# Autodesk Inventor assembly: LEFT RAIL ASSY
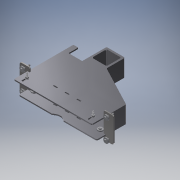
[picture p0: Inventor's stored thumbnail of the model, 180x180]
Saved by Autodesk Inventor 2018 (Build 220112000, 112)
## iProperties
Created: 2018-10-15
Part Number: LEFT RAIL ASSY
Material: Genérico
Document SubType Name: Assembly
Designer: Toshiba
Author: Toshiba
## Documents named in this file (7)
- C:\U\Semestre Primavera 2018\Diseño de sistemas mecánicos\CNC\DiseñoCNC\Gantry\LEFT RAIL ASSY.iam
- C:\U\Semestre Primavera 2018\Diseño de sistemas mecánicos\CNC\DiseñoCNC\Gantry\INTERNAL SIDE PLATE.ipt
- C:\U\Semestre Primavera 2018\Diseño de sistemas mecánicos\CNC\DiseñoCNC\Gantry\INTERNAL FRAME.ipt
- C:\U\Semestre Primavera 2018\Diseño de sistemas mecánicos\CNC\DiseñoCNC\Gantry\EXTERNAL SIDE PLATE.ipt
- C:\U\Semestre Primavera 2018\Diseño de sistemas mecánicos\CNC\DiseñoCNC\Gantry\SIDE BEARING GUIDE.ipt
- C:\U\Semestre Primavera 2018\Diseño de sistemas mecánicos\CNC\DiseñoCNC\Gantry\BEARING SYSTEM.iam
- C:\U\Semestre Primavera 2018\Diseño de sistemas mecánicos\CNC\DiseñoCNC\Gantry\FLANGE NUT M8.ipt
## Components (21 placed, 6 different names)
1. INTERNAL SIDE PLATE:1 — Coincidencia:1, Coincidencia:2, Coincidencia:3, Insertar:3, Insertar:4, Insertar:15, Insertar:16
2. INTERNAL FRAME:1 — Coincidencia:1, Coincidencia:2, Coincidencia:3, Coincidencia:4, Coincidencia:5, Coincidencia:6
3. EXTERNAL SIDE PLATE:1 — Coincidencia:4, Coincidencia:5, Coincidencia:6, Coincidencia:7, Nivelación:1, Coincidencia:8, Coincidencia:9, Insertar:7, Insertar:8, Insertar:11, Insertar:12
4. SIDE BEARING GUIDE:1 — Coincidencia:7, Nivelación:1, Coincidencia:8, Coincidencia:10, Insertar:5, Insertar:6, Insertar:9, Insertar:10
5. SIDE BEARING GUIDE:2 — Coincidencia:9, Coincidencia:10, Insertar:1, Insertar:2, Insertar:13, Insertar:14
6. BEARING SYSTEM:1 [sub-assembly] — Insertar:5
7. BEARING SYSTEM:2 [sub-assembly] — Insertar:6
8. BEARING SYSTEM:3 [sub-assembly] — Insertar:2
9. BEARING SYSTEM:4 [sub-assembly] — Insertar:1
10. BEARING SYSTEM:5 [sub-assembly] — Insertar:8
11. BEARING SYSTEM:6 [sub-assembly] — Insertar:7
12. BEARING SYSTEM:7 [sub-assembly] — Insertar:3
13. BEARING SYSTEM:8 [sub-assembly] — Insertar:4
14. FLANGE NUT M8:1 — Insertar:16
15. FLANGE NUT M8:2 — Insertar:15
16. FLANGE NUT M8:3 — Insertar:11
17. FLANGE NUT M8:4 — Insertar:12
18. FLANGE NUT M8:5 — Insertar:13
19. FLANGE NUT M8:6 — Insertar:14
20. FLANGE NUT M8:7 — Insertar:9
21. FLANGE NUT M8:8 — Insertar:10
## Relationships (27: Insert 16, Mate 10, Flush 1)
- Coincidencia:1 [Mate]: INTERNAL SIDE PLATE:1 ↔ INTERNAL FRAME:1
- Coincidencia:2 [Mate]: INTERNAL SIDE PLATE:1 ↔ INTERNAL FRAME:1
- Coincidencia:3 [Mate]: INTERNAL SIDE PLATE:1 ↔ INTERNAL FRAME:1
- Coincidencia:4 [Mate]: INTERNAL FRAME:1 ↔ EXTERNAL SIDE PLATE:1
- Coincidencia:5 [Mate]: INTERNAL FRAME:1 ↔ EXTERNAL SIDE PLATE:1
- Coincidencia:6 [Mate]: INTERNAL FRAME:1 ↔ EXTERNAL SIDE PLATE:1
- Coincidencia:7 [Mate]: EXTERNAL SIDE PLATE:1 ↔ SIDE BEARING GUIDE:1
- Nivelación:1 [Flush] (-21.5 mm): EXTERNAL SIDE PLATE:1 ↔ SIDE BEARING GUIDE:1
- Coincidencia:8 [Mate]: EXTERNAL SIDE PLATE:1 ↔ SIDE BEARING GUIDE:1
- Coincidencia:9 [Mate]: EXTERNAL SIDE PLATE:1 ↔ SIDE BEARING GUIDE:2
- Coincidencia:10 [Mate]: SIDE BEARING GUIDE:1 ↔ SIDE BEARING GUIDE:2
- Insertar:1 (5 mm): SIDE BEARING GUIDE:2 ↔ BEARING SYSTEM:4
- Insertar:2 (5 mm): SIDE BEARING GUIDE:2 ↔ BEARING SYSTEM:3
- Insertar:3: INTERNAL SIDE PLATE:1 ↔ BEARING SYSTEM:7
- Insertar:4: INTERNAL SIDE PLATE:1 ↔ BEARING SYSTEM:8
- Insertar:5 (5 mm): SIDE BEARING GUIDE:1 ↔ BEARING SYSTEM:1
- Insertar:6 (5 mm): SIDE BEARING GUIDE:1 ↔ BEARING SYSTEM:2
- Insertar:7: EXTERNAL SIDE PLATE:1 ↔ BEARING SYSTEM:6
- Insertar:8: EXTERNAL SIDE PLATE:1 ↔ BEARING SYSTEM:5
- Insertar:9: SIDE BEARING GUIDE:1 ↔ FLANGE NUT M8:7
- Insertar:10: SIDE BEARING GUIDE:1 ↔ FLANGE NUT M8:8
- Insertar:11: EXTERNAL SIDE PLATE:1 ↔ FLANGE NUT M8:3
- Insertar:12: EXTERNAL SIDE PLATE:1 ↔ FLANGE NUT M8:4
- Insertar:13: SIDE BEARING GUIDE:2 ↔ FLANGE NUT M8:5
- Insertar:14: SIDE BEARING GUIDE:2 ↔ FLANGE NUT M8:6
- Insertar:15: INTERNAL SIDE PLATE:1 ↔ FLANGE NUT M8:2
- Insertar:16: INTERNAL SIDE PLATE:1 ↔ FLANGE NUT M8:1
